# Autodesk Inventor assembly: Anglerfish
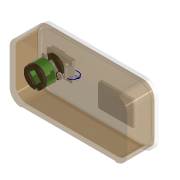
[picture p0: Inventor's stored thumbnail of the model, 180x180]
Saved by Autodesk Inventor 2022 (Build 260153000, 153)
## iProperties
Created: 2022-04-02
Part Number: Anglerfish
Document SubType Name: Assembly
Designer: Prakash Lab
Author: Prakash Lab
## Documents named in this file (9)
- C:\Users\diederichbenedict\Dropbox\Dokumente\Promotion\PROJECTS\Matchboxscope\INVENTOR\RELEASE\Anglerfish\Workspace\Anglerfish.iam
- C:\Users\diederichbenedict\Dropbox\Dokumente\Promotion\PROJECTS\Matchboxscope\INVENTOR\RELEASE\Anglerfish\Workspace\00_Powerbank.ipt
- C:\Users\diederichbenedict\Dropbox\Dokumente\Promotion\PROJECTS\Matchboxscope\INVENTOR\RELEASE\Anglerfish\Workspace\00_lunchbox_body.ipt
- C:\Users\diederichbenedict\Dropbox\Dokumente\Promotion\PROJECTS\Matchboxscope\INVENTOR\RELEASE\Anglerfish\Workspace\00_Lunchbox_cover.ipt
- C:\Users\diederichbenedict\Dropbox\Dokumente\Promotion\PROJECTS\Matchboxscope\INVENTOR\RELEASE\Anglerfish\Workspace\Anglerfish_coverslipclamp_top.ipt
- C:\Users\diederichbenedict\Dropbox\Dokumente\Promotion\PROJECTS\Matchboxscope\INVENTOR\RELEASE\Anglerfish\Workspace\Anglerfish_coverslipclamp_levelarm.ipt
- C:\Users\diederichbenedict\Dropbox\Dokumente\Promotion\PROJECTS\Matchboxscope\INVENTOR\RELEASE\Anglerfish\Workspace\Anglerfish_coverslipclamp_lampclamp.ipt
- C:\Users\diederichbenedict\Dropbox\Dokumente\Promotion\PROJECTS\Matchboxscope\INVENTOR\RELEASE\InjectionMolded\Assembly_Matchboxscope_injectionmolded_Anglerfish.iam
- C:\Users\diederichbenedict\Dropbox\Dokumente\Promotion\PROJECTS\Matchboxscope\INVENTOR\RELEASE\InjectionMolded\00_LED_lamp.ipt
## Components (9 placed, 8 different names)
1. 00_Powerbank:1
2. 00_lunchbox_body:1 — Fluchtend:4, Winkel:14, Fluchtend:33, Fluchtend:34, Passend:31
3. 00_Lunchbox_cover:1 — Fluchtend:33, Fluchtend:34, Passend:31, Passend:32, Winkel:15, Passend:34
4. 00_Powerbank:2
5. Anglerfish_coverslipclamp_top:1 — Fluchtend:36, Fluchtend:37, Fluchtend:38, Fluchtend:39, Passend:32, Winkel:15
6. Anglerfish_coverslipclamp_levelarm:1 — Fluchtend:36, Fluchtend:37
7. Anglerfish_coverslipclamp_lampclamp:1 — Fluchtend:38, Fluchtend:39, Passend:33, Einfügen:1
8. Assembly_Matchboxscope_injectionmolded_Anglerfish:1 [sub-assembly] — Passend:33, Passend:34
9. 00_LED_lamp:1 — Einfügen:1
## Relationships (14: Flush 7, Mate 4, Angle 2, Insert 1)
- Fluchtend:4 [Flush]: 00_lunchbox_body:1
- Winkel:14 [Angle] (180 deg): 00_lunchbox_body:1
- Fluchtend:33 [Flush]: 00_lunchbox_body:1 ↔ 00_Lunchbox_cover:1
- Fluchtend:34 [Flush]: 00_lunchbox_body:1 ↔ 00_Lunchbox_cover:1
- Passend:31 [Mate]: 00_lunchbox_body:1 ↔ 00_Lunchbox_cover:1
- Fluchtend:36 [Flush]: Anglerfish_coverslipclamp_top:1 ↔ Anglerfish_coverslipclamp_levelarm:1
- Fluchtend:37 [Flush]: Anglerfish_coverslipclamp_top:1 ↔ Anglerfish_coverslipclamp_levelarm:1
- Fluchtend:38 [Flush]: Anglerfish_coverslipclamp_top:1 ↔ Anglerfish_coverslipclamp_lampclamp:1
- Fluchtend:39 [Flush]: Anglerfish_coverslipclamp_top:1 ↔ Anglerfish_coverslipclamp_lampclamp:1
- Passend:32 [Mate]: 00_Lunchbox_cover:1 ↔ Anglerfish_coverslipclamp_top:1
- Winkel:15 [Angle] (0 deg): 00_Lunchbox_cover:1 ↔ Anglerfish_coverslipclamp_top:1
- Passend:33 [Mate]: Anglerfish_coverslipclamp_lampclamp:1 ↔ Assembly_Matchboxscope_injectionmolded_Anglerfish:1
- Passend:34 [Mate]: 00_Lunchbox_cover:1 ↔ Assembly_Matchboxscope_injectionmolded_Anglerfish:1
- Einfügen:1 [Insert]: Anglerfish_coverslipclamp_lampclamp:1 ↔ 00_LED_lamp:1
